# Autodesk Inventor assembly: FullUnitMockup
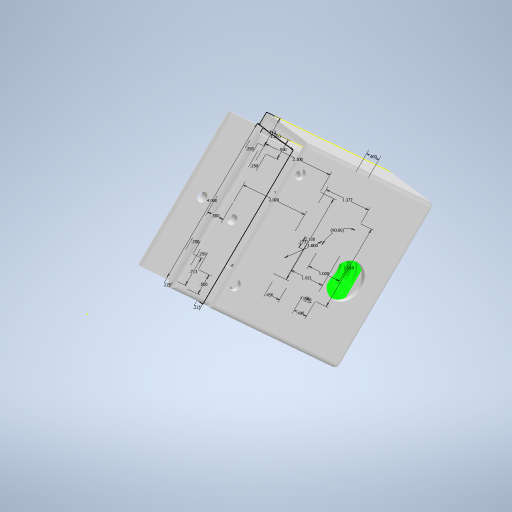
[picture p0: Inventor's stored thumbnail of the model, 512x512]
Saved by Autodesk Inventor 2024.1 (Build 281209000, 209)
## iProperties
Created: 2024-08-21
Part Number: FullUnitMockup
Document SubType Name: Assembly
Designer: pab2
Author: pab2
## Documents named in this file (5)
- C:\Users\pab2\Documents\GitHub\AFL-hardware-devel\Instrument-Interfacing\SANS ThermalBlock\FullUnitMockup.iam
- C:\Users\pab2\Documents\GitHub\AFL-hardware-devel\Instrument-Interfacing\SANS ThermalBlock\Al thermal core.ipt
- C:\Users\pab2\Documents\GitHub\AFL-hardware-devel\Instrument-Interfacing\SANS ThermalBlock\Rail Clip.ipt
- C:\Users\pab2\Documents\GitHub\AFL-hardware-devel\Instrument-Interfacing\NCNR SANS\2 mm Ti cell - for machining.ipt
- C:\Users\pab2\Documents\GitHub\AFL-hardware-devel\Instrument-Interfacing\SANS ThermalBlock\ThermalOvershield.ipt
## Components (4 placed, 4 different names)
1. Al thermal core:1 — Mate:1, Mate:2, Mate:3, Mate:4, Mate:5, Mate:8
2. Rail Clip:1 — Mate:1, Mate:2, Mate:5, Mate:6, Mate:7
3. 2 mm Ti cell - for machining:1 — Mate:3, Mate:4
4. ThermalOvershield:1 — Mate:6, Mate:7, Mate:8
## Relationships (8: Mate 8)
- Mate:1: Al thermal core:1 ↔ Rail Clip:1
- Mate:2: Al thermal core:1 ↔ Rail Clip:1
- Mate:3: Al thermal core:1 ↔ 2 mm Ti cell - for machining:1
- Mate:4: Al thermal core:1 ↔ 2 mm Ti cell - for machining:1
- Mate:5: Al thermal core:1 ↔ Rail Clip:1
- Mate:6: Rail Clip:1 ↔ ThermalOvershield:1
- Mate:7: Rail Clip:1 ↔ ThermalOvershield:1
- Mate:8: Al thermal core:1 ↔ ThermalOvershield:1
